# Autodesk Inventor assembly: Arm Rod
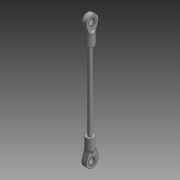
[picture p0: Inventor's stored thumbnail of the model, 180x180]
Saved by Autodesk Inventor 2014 SP1 (Build 180222100, 222)
## iProperties
Created: 2013-12-29
Part Number: Arm Rod
Document SubType Name: Assembly
Designer: tom
Author: tom
## Documents named in this file (3)
- C:\Users\tom\Documents\GitHub\Delta_Robots\Delatabot - Small Model\Inventor\Deltabot - Small Model\Arm Rod.iam
- C:\Users\tom\Documents\GitHub\Delta_Robots\Delatabot - Small Model\Inventor\Deltabot - Small Model\Body.ipt
- C:\Users\tom\Documents\GitHub\Vacubot\Inventor\Arm Rod.ipt
## Components (3 placed, 2 different names)
1. Body:1
2. Rod
3. Body:2
## Relationships (4: Mate 4)
- [Mate]: Body:1 ↔ Rod
- [Mate]: Body:1 ↔ Rod
- [Mate]: Rod ↔ Body:2
- [Mate]: Rod ↔ Body:2
